# Autodesk Inventor assembly: gun assemble v1
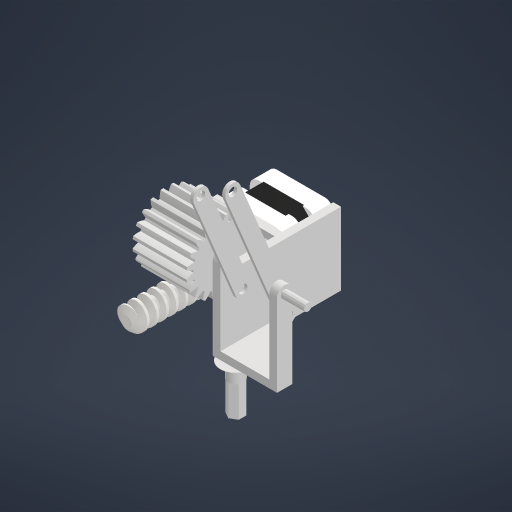
[picture p0: Inventor's stored thumbnail of the model, 512x512]
Saved by Autodesk Inventor 2024 (Build 280153000, 153)
## iProperties
Created: 2023-06-18
Part Number: gun assemble v1
Document SubType Name: Assembly
Designer: 6gioc
Mass: 183.788 g
Surface Area: 588.653 cm^2
Volume: 135.53 cm^3
Density: 1.35607 g/cm^3
Author: 6gioc
## Documents named in this file (8)
- C:\Users\wodyd\Downloads\AAST\PART\AAST Main\gun assemble v1.iam
- C:\Users\wodyd\Downloads\AAST\PART\AAST Main\gunholder_clip v2.ipt
- C:\Users\wodyd\Downloads\AAST\PART\AAST Main\stepmotor v1.ipt
- C:\Users\wodyd\Downloads\AAST\PART\AAST Main\worm.iam
- C:\Users\wodyd\Downloads\AAST\PART\AAST Main\m10 washa.ipt
- C:\Users\wodyd\Downloads\AAST\PART\AAST Main\gunholder_v3 L.ipt
- C:\Users\wodyd\Downloads\AAST\PART\AAST Main\gunholder_v3 R.ipt
- C:\Users\wodyd\Downloads\AAST\PART\AAST Main\30mm_gear_hexagon.iam
## Components (7 placed, 7 different names)
1. gunholder_clip v2:1 — 회전:2, 회전:3, 회전:4, 강체:5
2. stepmotor v1:1 — 강체:5, 회전:5
3. worm:1 [sub-assembly] — 회전:5, 회전:1
4. m10 washa:1 — 회전:2
5. gunholder_v3 L:1 — 회전:3, 회전:2
6. gunholder_v3 R:1 — 회전:4, 강체:4, 회전:1, 회전:2
7. 30mm_gear_hexagon:1 [sub-assembly] — 강체:4
## Relationships (8: RevoluteJoint 4, WeldJoint 2, RelateRotation 2)
- 회전:2 [RevoluteJoint]: gunholder_clip v2:1 ↔ m10 washa:1
- 회전:3 [RevoluteJoint]: gunholder_clip v2:1 ↔ gunholder_v3 L:1
- 회전:4 [RevoluteJoint]: gunholder_clip v2:1 ↔ gunholder_v3 R:1
- 강체:4 [WeldJoint]: gunholder_v3 R:1 ↔ 30mm_gear_hexagon:1
- 강체:5 [WeldJoint]: gunholder_clip v2:1 ↔ stepmotor v1:1
- 회전:5 [RevoluteJoint]: stepmotor v1:1 ↔ worm:1
- 회전:1 [RelateRotation] (-20 ul): worm:1 ↔ gunholder_v3 R:1
- 회전:2 [RelateRotation] (1 ul): gunholder_v3 L:1 ↔ gunholder_v3 R:1
